# Autodesk Inventor assembly: 36T_idler
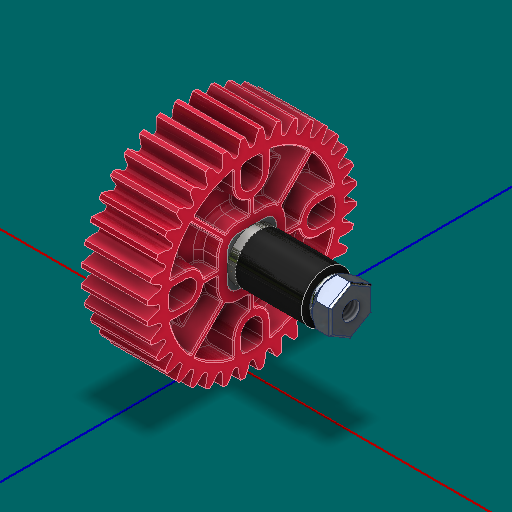
[picture p0: Inventor's stored thumbnail of the model, 512x512]
Saved by Autodesk Inventor 2025 (Build 290162000, 162)
## iProperties
Created: 2024-08-19
Part Number: 36T_idler
Document SubType Name: Assembly
Designer: averey
Author: averey
## Documents named in this file (8)
- C:\Users\avere\vex_robotics_high_stakes\hardware\cad\ATLAS\tower\intake_gearbox\36T_idler.iam
- C:\Users\avere\vex_robotics_high_stakes\hardware\cad\VEX-CAD-Inventor\Motion\Gears\HS Gear\HS 36T Gear, No Insert.iam
- C:\Users\avere\vex_robotics_high_stakes\hardware\cad\VEX-CAD-Inventor\Motion\Gears\HS Gear.iam
- C:\Users\avere\vex_robotics_high_stakes\hardware\cad\VEX-CAD-Inventor\Structure\Hardware\Nut Thin Nylock.ipt
- C:\Users\avere\vex_robotics_high_stakes\hardware\cad\VEX-CAD-Inventor\Motion\Spacers\Spacer Nylon .375 OD.ipt
- C:\Users\avere\vex_robotics_high_stakes\hardware\cad\VEX-CAD-Inventor\Motion\Spacers\Spacer Nylon .375 OD\NSpacer .375 OD x .500.ipt
- C:\Users\avere\vex_robotics_high_stakes\hardware\cad\VEX-CAD-Inventor\Motion\Spacers\Washer Steel\SWasher .375 OD x .062500.ipt
- C:\Users\avere\vex_robotics_high_stakes\hardware\cad\VEX-CAD-Inventor\Motion\Spacers\Washer Steel.ipt
## Components (5 placed, 4 different names)
1. HS 36T Gear, No Insert:2 [sub-assembly] — Insert:4, Insert:7
2. Nut Thin Nylock:1 — Insert:3
3. NSpacer .375 OD x .500:2 — Insert:3, Insert:6
4. Nut Thin Nylock:2 — Insert:4
5. SWasher .375 OD x .062500:1 — Insert:6, Insert:7
## Relationships (4: Insert 4)
- Insert:3: Nut Thin Nylock:1 ↔ NSpacer .375 OD x .500:2
- Insert:4: HS 36T Gear, No Insert:2 ↔ Nut Thin Nylock:2
- Insert:6: NSpacer .375 OD x .500:2 ↔ SWasher .375 OD x .062500:1
- Insert:7: HS 36T Gear, No Insert:2 ↔ SWasher .375 OD x .062500:1
